# Autodesk Inventor assembly: Drive
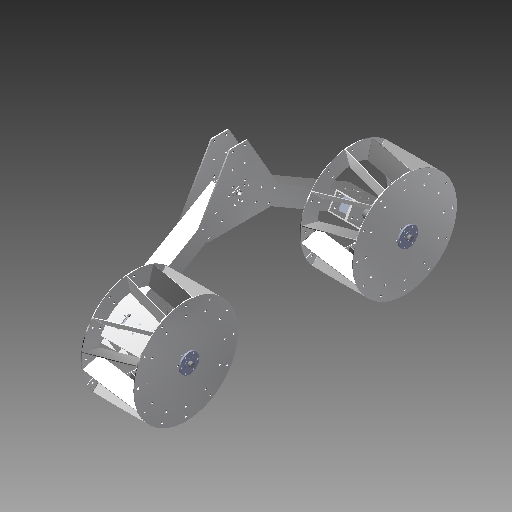
[picture p0: Inventor's stored thumbnail of the model, 512x512]
Saved by Autodesk Inventor 2019 (Build 230136000, 136)
## iProperties
Created: 2018-10-29
Part Number: Drive
Document SubType Name: Assembly
Designer: Adhik
Author: Adhik
## Documents named in this file (4)
- C:\Users\mcgowc2\Desktop\Rock Raiders\Chassis_Final\Drive.iam
- C:\Users\mcgowc2\Desktop\Rock Raiders\Chassis_Final\Gusset Plate.ipt
- C:\Users\mcgowc2\Desktop\Rock Raiders\Chassis_Final\Drive Arm.iam
- C:\Users\mcgowc2\Desktop\Rock Raiders\Chassis_Final\Arm Bearing.ipt
## Components (6 placed, 3 different names)
1. Gusset Plate:1 — Mate:1, Mate:2, Mate:3, Mate:4, Mate:5, Mate:6, Insert:1
2. Gusset Plate:2 — Mate:7, Mate:8, Mate:9, Insert:2
3. Drive Arm:1 [sub-assembly] — Mate:1, Mate:3, Mate:4, Mate:9
4. Drive Arm:2 [sub-assembly] — Mate:2, Mate:5, Mate:6, Mate:7, Mate:8
5. Arm Bearing:1 — Insert:1
6. Arm Bearing:2 — Insert:2
## Relationships (11: Mate 9, Insert 2)
- Mate:1: Gusset Plate:1 ↔ Drive Arm:1
- Mate:2: Gusset Plate:1 ↔ Drive Arm:2
- Mate:3: Gusset Plate:1 ↔ Drive Arm:1
- Mate:4: Gusset Plate:1 ↔ Drive Arm:1
- Mate:5: Gusset Plate:1 ↔ Drive Arm:2
- Mate:6: Gusset Plate:1 ↔ Drive Arm:2
- Mate:7: Gusset Plate:2 ↔ Drive Arm:2
- Mate:8: Gusset Plate:2 ↔ Drive Arm:2
- Mate:9: Gusset Plate:2 ↔ Drive Arm:1
- Insert:1: Gusset Plate:1 ↔ Arm Bearing:1
- Insert:2: Gusset Plate:2 ↔ Arm Bearing:2
